# Autodesk Inventor assembly: Roll_Fixation_Set
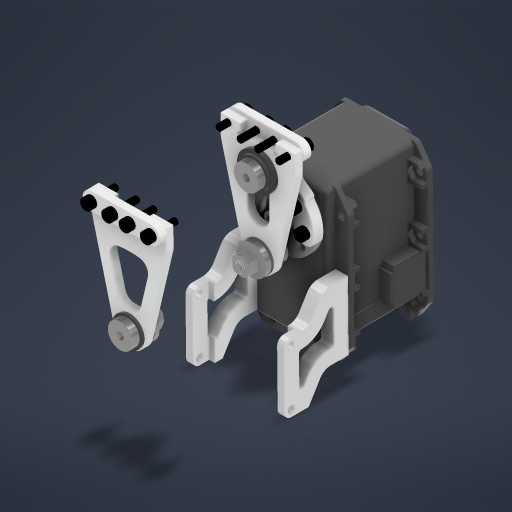
[picture p0: Inventor's stored thumbnail of the model, 512x512]
Saved by Autodesk Inventor 2024.3 (Build 283343000, 343)
## iProperties
Created: 2024-02-15
Part Number: Roll_Fixation_Set
Document SubType Name: Assembly
Designer: ASUS
Author: ASUS
## Documents named in this file (16)
- C:\Users\ASUS\Desktop\Anti_Backlash_Structure_OP\v4_Frame\Roll_Fixation_Set.iam
- C:\Users\ASUS\Desktop\Anti_Backlash_Structure_OP\v4_Frame\Roll_Fixation_Frame.ipt
- C:\Users\ASUS\Desktop\Anti_Backlash_Structure_OP\v4_Frame\Roll_Fixation_Frame_Back.ipt
- C:\Users\ASUS\Desktop\Anti_Backlash_Structure_OP\v4_Frame\hip joint fix washer.ipt
- C:\Users\ASUS\Desktop\Anti_Backlash_Structure_OP\MISUMI\hip_joint_fix_washer_10mm_Set.iam
- C:\Users\ASUS\Desktop\Anti_Backlash_Structure_OP\v4_Frame\Front_Frame_Fixer_v2.iam
- C:\Users\ASUS\Desktop\Anti_Backlash_Structure_OP\ROBOTIS(Inventor 2024 ver.)\DXL\MX-64T.ipt
- C:\Users\ASUS\Desktop\Anti_Backlash_Structure_OP\MISUMI\DBSY4-5-8.ipt
- C:\Users\ASUS\Desktop\Anti_Backlash_Structure_OP\MISUMI\LED-0606.ipt
- C:\Users\ASUS\Desktop\Anti_Backlash_Structure_OP\v4_Frame\Ubber_Washer_1.5mm.ipt
- C:\Users\ASUS\Desktop\Anti_Backlash_Structure_OP\MISUMI\DBB4-8-5.ipt
- C:\Users\ASUS\Desktop\Anti_Backlash_Structure_OP\MISUMI\NBW-0612-10.ipt
- C:\Users\ASUS\Desktop\Anti_Backlash_Structure_OP\MISUMI\C-WSSA12-4-2.ipt
- C:\Users\ASUS\Desktop\Anti_Backlash_Structure_OP\v4_Frame\ABD_Slider_Set_v4.iam
- C:\Users\ASUS\Desktop\Anti_Backlash_Structure_OP\v4_Frame\Dynamixel Vertical fixation.ipt
- C:\Users\ASUS\Desktop\Anti_Backlash_Structure_OP\v4_Frame\Dynamixel Vertical fixation_MIR.ipt
## Components (20 placed, 15 different names)
1. Roll_Fixation_Frame:2 — 메이트:27
2. hip joint fix washer:3
3. hip joint fix washer:4
4. hip_joint_fix_washer_10mm_Set:3 [sub-assembly] — 메이트:28, 메이트:29
5. hip_joint_fix_washer_10mm_Set:4 [sub-assembly] — 메이트:28, 메이트:29, 메이트:33
6. Front_Frame_Fixer_v2:2 [sub-assembly]
7. DBSY4-5-8:2 — 메이트:32
8. MX-64T:2 — 메이트:31, 각도:1
9. LED-0606:1
10. Ubber_Washer_1.5mm:1
11. DBB4-8-5:1
12. NBW-0612-10:1
13. C-WSSA12-4-2:1
14. NBW-0612-10:2
15. ABD_Slider_Set_v4:1 [sub-assembly] — 메이트:30
16. Roll_Fixation_Frame_Back:2 — 메이트:27, 메이트:33, 각도:1
17. Dynamixel Vertical fixation:1
18. Dynamixel Vertical fixation_MIR:1
19. Front_Frame_Fixer_v2:3 [sub-assembly] — 메이트:30, 메이트:31, 메이트:32
20. DBSY4-5-8:3
## Relationships (38: Mate 20, Insert 17, Angle 1)
- [Insert]: Roll_Fixation_Frame:2 ↔ hip joint fix washer:3
- [Insert]: Roll_Fixation_Frame:2 ↔ hip joint fix washer:3
- [Mate]: Roll_Fixation_Frame:2 ↔ hip joint fix washer:3
- [Insert]: hip joint fix washer:3 ↔ hip_joint_fix_washer_10mm_Set:3
- [Mate]: hip joint fix washer:3 ↔ hip_joint_fix_washer_10mm_Set:3
- [Insert]: hip joint fix washer:4 ↔ hip_joint_fix_washer_10mm_Set:4
- [Mate]: hip joint fix washer:4 ↔ hip_joint_fix_washer_10mm_Set:4
- [Mate]: hip_joint_fix_washer_10mm_Set:3 ↔ hip_joint_fix_washer_10mm_Set:4
- [Mate]: hip_joint_fix_washer_10mm_Set:3 ↔ hip_joint_fix_washer_10mm_Set:4
- [Insert]: Front_Frame_Fixer_v2:2 ↔ DBSY4-5-8:2
- [Insert]: Roll_Fixation_Frame:2 ↔ Front_Frame_Fixer_v2:2
- [Insert]: LED-0606:1 ↔ Ubber_Washer_1.5mm:1
- [Insert]: Ubber_Washer_1.5mm:1 ↔ NBW-0612-10:2
- [Insert]: DBB4-8-5:1 ↔ NBW-0612-10:2
- [Insert]: NBW-0612-10:1 ↔ C-WSSA12-4-2:1
- [Mate]: DBB4-8-5:1 ↔ ABD_Slider_Set_v4:1
- [Insert]: LED-0606:1 ↔ NBW-0612-10:1
- [Insert]: C-WSSA12-4-2:1 ↔ ABD_Slider_Set_v4:1
- [Insert] (0.5 mm): MX-64T:2 ↔ ABD_Slider_Set_v4:1
- [Mate]: Ubber_Washer_1.5mm:1 ↔ Roll_Fixation_Frame_Back:2
- [Insert]: hip joint fix washer:4 ↔ Roll_Fixation_Frame_Back:2
- [Mate]: hip joint fix washer:4 ↔ hip_joint_fix_washer_10mm_Set:4
- [Mate]: MX-64T:2 ↔ Dynamixel Vertical fixation:1
- [Mate]: MX-64T:2 ↔ Dynamixel Vertical fixation:1
- [Mate]: MX-64T:2 ↔ Dynamixel Vertical fixation:1
- [Insert]: MX-64T:2 ↔ Dynamixel Vertical fixation_MIR:1
- [Mate]: MX-64T:2 ↔ Dynamixel Vertical fixation_MIR:1
- [Mate] (0.5 mm): LED-0606:1 ↔ Roll_Fixation_Frame_Back:2
- [Insert]: Front_Frame_Fixer_v2:3 ↔ DBSY4-5-8:3
- [Insert]: Roll_Fixation_Frame_Back:2 ↔ Front_Frame_Fixer_v2:3
- 메이트:27 [Mate] (49 mm): Roll_Fixation_Frame:2 ↔ Roll_Fixation_Frame_Back:2
- 메이트:28 [Mate]: hip_joint_fix_washer_10mm_Set:3 ↔ hip_joint_fix_washer_10mm_Set:4
- 메이트:29 [Mate]: hip_joint_fix_washer_10mm_Set:3 ↔ hip_joint_fix_washer_10mm_Set:4
- 메이트:30 [Mate] (10 mm): ABD_Slider_Set_v4:1 ↔ Front_Frame_Fixer_v2:3
- 메이트:31 [Mate] (-14.5 mm): MX-64T:2 ↔ Front_Frame_Fixer_v2:3
- 메이트:32 [Mate]: DBSY4-5-8:2 ↔ Front_Frame_Fixer_v2:3
- 메이트:33 [Mate]: hip_joint_fix_washer_10mm_Set:4 ↔ Roll_Fixation_Frame_Back:2
- 각도:1 [Angle] (0 deg): MX-64T:2 ↔ Roll_Fixation_Frame_Back:2
## Named parameters: d1047_d49 = 0 mm, d71_d49 = 0 mm, d72_d50 = 0 mm, d73_d17 = 0 mm, d74_d18 = 0 mm, d75_d838 = 0 mm, d76_d839 = 0 mm, d77_d840 = 0 mm, d78_d841 = 0 mm, d79_d753 = 0 mm, d80_d754 = 0 mm, d81_d764 = 0 mm, d1010_d968 = 0 mm, d1011_d969 = 0 mm, d1012_d971 = 0 mm, d1013_d941 = 0 mm, d1014_d956 = 0 mm, d1015_d957 = 0 mm, d1016_d960 = 0 mm
